# Autodesk Inventor assembly: Cutout Bottom
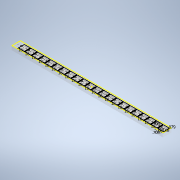
[picture p0: Inventor's stored thumbnail of the model, 180x180]
Saved by Autodesk Inventor 2022 (Build 260153000, 153)
## iProperties
Created: 2022-03-03
Part Number: Cutout Bottom
Document SubType Name: Assembly
Designer: Nathan Griffith
Author: Nathan Griffith
## Documents named in this file (4)
- C:\Users\Nathan Griffith\Documents\Inventor\Eric's Keyboard\Cutout Bottom.iam
- C:\Users\Nathan Griffith\Documents\Inventor\Eric's Keyboard\Stock.ipt
- C:\Users\Nathan Griffith\Documents\Inventor\Eric's Keyboard\Keycap.ipt
- C:\Users\Nathan Griffith\Documents\Inventor\Eric's Keyboard\Template Placement.ipt
## Components (24 placed, 3 different names)
1. Stock:1 — Mate:1, Mate:2, Mate:3
2. Template Placement:1 — Mate:1, Mate:2, Mate:3, Mate:4, Mate:5, Mate:6
3. Keycap:1 — Mate:4, Mate:5, Mate:6
4. Keycap:2
5. Keycap:3
6. Keycap:4
7. Keycap:5
8. Keycap:6
9. Keycap:7
10. Keycap:8
11. Keycap:9
12. Keycap:10
13. Keycap:11
14. Keycap:12
15. Keycap:13
16. Keycap:14
17. Keycap:15
18. Keycap:16
19. Keycap:17
20. Keycap:18
21. Keycap:19
22. Keycap:20
23. Keycap:21
24. Keycap:22
## Component patterns: (22 elements, first: Keycap:1)
## Relationships (6: Mate 6)
- Mate:1: Stock:1 ↔ Template Placement:1
- Mate:2: Stock:1 ↔ Template Placement:1
- Mate:3: Stock:1 ↔ Template Placement:1
- Mate:4: Template Placement:1 ↔ Keycap:1
- Mate:5: Template Placement:1 ↔ Keycap:1
- Mate:6: Template Placement:1 ↔ Keycap:1
